# Autodesk Inventor assembly: WormGearExperiementWithClutch
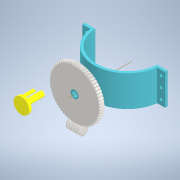
[picture p0: Inventor's stored thumbnail of the model, 180x180]
Saved by Autodesk Inventor 2021 (Build 250183000, 183)
## iProperties
Created: 2020-06-28
Part Number: WormGearExperiementWithClutch
Document SubType Name: Assembly
Designer: robst
Author: robst
## Documents named in this file (4)
- C:\git\CAD-Development\robSteele\ShapeWays\TelescopeProjects\TelescopeMount\WormGearExperiementWithClutch.iam
- C:\git\CAD-Development\robSteele\ShapeWays\TelescopeProjects\TelescopeMount\ForkMountWith6inchBevelGear\Design Accelerator\Worm Gears2.iam
- C:\git\CAD-Development\robSteele\ShapeWays\TelescopeProjects\TelescopeMount\tubeBracketV02.ipt
- C:\git\CAD-Development\robSteele\ShapeWays\TelescopeProjects\TelescopeMount\innerClutch.ipt
## Components (3 placed, 3 different names)
1. Worm Gears:1 [sub-assembly] — Insert:1
2. tubeBracketV02:1 — Insert:1
3. innerClutch:1
## Relationships (1: Insert 1)
- Insert:1: Worm Gears:1 ↔ tubeBracketV02:1
